# Autodesk Inventor assembly: Bearing-Pillow-Block-Short-Through-Bore
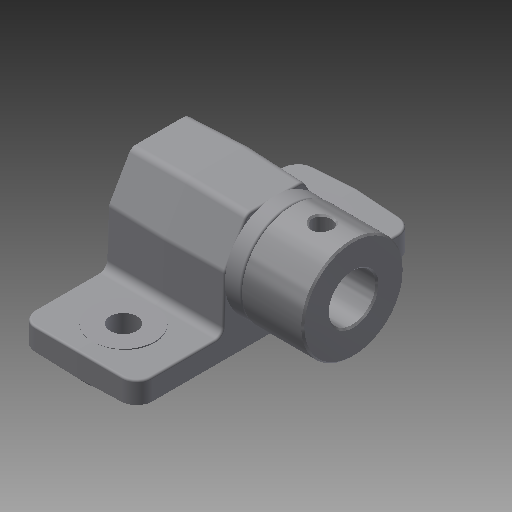
[picture p0: Inventor's stored thumbnail of the model, 512x512]
Saved by Autodesk Inventor 2017.3 (Build 213256000, 256)
## iProperties
Created: 2018-01-05
Part Number: Bearing-Pillow-Block-Short-Through-Bore
Document SubType Name: Assembly
Designer: pranav
Author: pranav
## iProperties of the stored document REV-41-1326.ipt
Created: 2016-09-04
Part Number: REV-41-1326
Material: Generic
Description: STEP AP203
Document SubType Name: Modeling
Designer: pranav
Density: 1 g/cm^3
Appearance: Default
Sending System: SolidWorks 2015
Preprocessor: SwSTEP 2.0
Title: REV-41-1326_Default.step
Revision Number: ANY
## iProperties of the stored document REV-41-1327.ipt
Created: 2017-04-10
Part Number: REV-41-1327
Material: Generic
Document SubType Name: Modeling
Designer: pranav
Density: 1 g/cm^3
Appearance: Default
Sending System: Autodesk Translation Framework v5.2.0.2920
Preprocessor: ST-DEVELOPER v16.5
Title: E:/Dropbox/REV Robotics/STEP Files/REV-41-1327.step
## iProperties of the stored document REV-41-1317.ipt
Created: 2016-09-04
Part Number: REV-41-1317
Material: Generic
Description: STEP AP203
Document SubType Name: Modeling
Designer: pranav
Density: 1 g/cm^3
Appearance: Default
Sending System: SolidWorks 2015
Preprocessor: SwSTEP 2.0
Title: REV-41-1317_Default.step
Revision Number: ANY
## Documents named in this file (7)
- **C:\Users\pranav\Documents\Inventor\REV-Robot-CAD\Bearing-Pillow-Block-Short-Through-Bore.iam*LocalDocs*xF1s5e1j1Ypn1upgvWnj31za4Yh*REV-41-1326.ipt
- **C:\Users\pranav\Documents\Inventor\REV-Robot-CAD\Bearing-Pillow-Block-Short-Through-Bore.iam*LocalDocs*xDyqmxhlnGwede0s4Lpzfnq5gLd*REV-41-1327.ipt
- **C:\Users\pranav\Documents\Inventor\REV-Robot-CAD\Bearing-Pillow-Block-Short-Through-Bore.iam*LocalDocs*xUpebkwetHcibu5cpIn2ahq2oQd*REV-41-1317.ipt
- C:\Users\pranav\Documents\Inventor\REV-Robot-CAD\Bearing-Pillow-Block-Short-Through-Bore.iam
- C:\Users\pranav\Documents\Inventor\REV-Robot-CAD\REV Robotics\REV Robotics CAD\REV-41-1317.step
- C:\Users\pranav\Documents\Inventor\REV-Robot-CAD\REV Robotics\REV Robotics CAD\REV-41-1326.step
- C:\Users\pranav\Documents\Inventor\REV-Robot-CAD\REV Robotics\REV Robotics CAD\REV-41-1327.step
## Components (3 placed, 3 different names)
1. REV-41-1317:1 — Mate:2, Mate:3, Mate:5
2. REV-41-1326:1 — Mate:2, Mate:3, Mate:4
3. REV-41-1327:1 — Mate:4, Mate:5
## Relationships (4: Mate 4)
- Mate:2: REV-41-1317:1 ↔ REV-41-1326:1
- Mate:3: REV-41-1317:1 ↔ REV-41-1326:1
- Mate:4: REV-41-1326:1 ↔ REV-41-1327:1
- Mate:5: REV-41-1317:1 ↔ REV-41-1327:1
